# Autodesk Inventor assembly: STK00-000
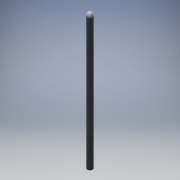
[picture p0: Inventor's stored thumbnail of the model, 180x180]
Saved by Autodesk Inventor 2018 (Build 220112000, 112)
## iProperties
Created: 2018-02-13
Part Number: STK00-000
Document SubType Name: Assembly
Designer: JARVIS
Author: JARVIS
## Documents named in this file (4)
- D:\Smartgit\Hobby\FlowSensorV2.1\STK00-000.iam
- D:\Smartgit\Hobby\FlowSensorV2.1\STK00-001.ipt
- D:\Smartgit\Hobby\FlowSensorV2.1\STK00-002.ipt
- D:\Smartgit\Hobby\FlowSensorV2.1\STK00-003.ipt
## Components (3 placed, 3 different names)
1. STK00-002:1 — Mate:1, Mate:3, Tangent:1
2. STK00-001:1 — Mate:1
3. STK00-003:1 — Mate:3, Tangent:1
## Relationships (3: Mate 2, Tangent 1)
- Mate:1: STK00-002:1 ↔ STK00-001:1
- Mate:3: STK00-002:1 ↔ STK00-003:1
- Tangent:1: STK00-002:1 ↔ STK00-003:1
